# Autodesk Inventor assembly: 0401 ASY GBK wall shield Center 1
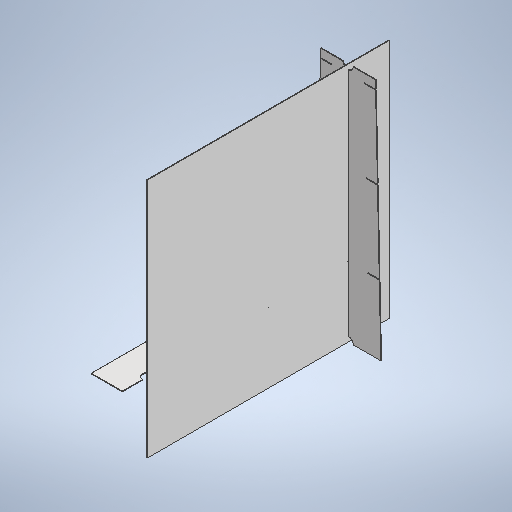
[picture p0: Inventor's stored thumbnail of the model, 512x512]
Saved by Autodesk Inventor 2026.2 (Build 302298000, 298)
## iProperties
Created: 2026-05-19
Part Number: 0401 ASY GBK wall shield Center 1
Document SubType Name: Assembly
Designer: admin
Author: admin
## Documents named in this file (4)
- C:\Users\admin\Documents\Inventor\GBK-Gubkinskiy\0401 ASY GBK wall shield Center 1.iam
- C:\Users\admin\Documents\Inventor\GBK-Gubkinskiy\0411 GBK Center main rib.ipt
- C:\Users\admin\Documents\Inventor\GBK-Gubkinskiy\0413 GBK stringer C1.ipt
- C:\Users\admin\Documents\Inventor\GBK-Gubkinskiy\01.1 GBK shield.ipt
## Components (4 placed, 3 different names)
1. 0411 GBK Center main rib:1 — Rigid:1, Flush:3, Mate:5, Flush:4, Flush:5
2. 0413 GBK stringer C1:1 — Rigid:1
3. Part111:1 — Mate:1, Flush:1, Mate:2, Flush:2, Mate:4, Flush:3, Mate:5, Flush:5
4. 0411 GBK Center main rib:2 — Flush:2, Mate:4, Flush:4
## Relationships (10: Flush 5, Mate 4, WeldJoint 1)
- Rigid:1 [WeldJoint] (4 mm): 0411 GBK Center main rib:1 ↔ 0413 GBK stringer C1:1
- Mate:1: Part111:1
- Flush:1: Part111:1
- Mate:2: Part111:1
- Flush:2: Part111:1 ↔ 0411 GBK Center main rib:2
- Mate:4: Part111:1 ↔ 0411 GBK Center main rib:2
- Flush:3: 0411 GBK Center main rib:1 ↔ Part111:1
- Mate:5: 0411 GBK Center main rib:1 ↔ Part111:1
- Flush:4: 0411 GBK Center main rib:1 ↔ 0411 GBK Center main rib:2
- Flush:5 (250 mm): 0411 GBK Center main rib:1 ↔ Part111:1
